# Autodesk Inventor assembly: ASY МОО 001 отстойник осветлитель
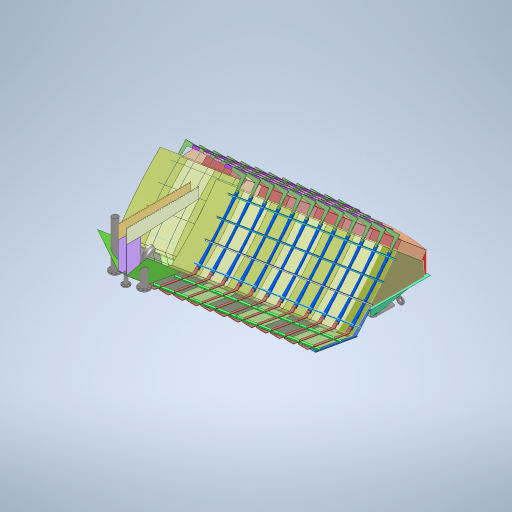
[picture p0: Inventor's stored thumbnail of the model, 512x512]
Saved by Autodesk Inventor 2024.2 (Build 282272000, 272)
## iProperties
Created: 2024-04-28
Part Number: ASY МОО 001 отстойник осветлитель
Document SubType Name: Weldment
Designer: admin
Weld Material: Welded Aluminum-6061
Mass: 1.58517e+06 g
Surface Area: 1.48953e+06 cm^2
Volume: 226523 cm^3
Density: 6.99781 g/cm^3
Author: admin
## Documents named in this file (40)
- C:\Users\pokla\Documents\Inventor\Отстойник осветлитель\Manturovo_Se-clar-Gleb\ASY МОО 001 отстойник осветлитель.iam
- C:\Users\pokla\Documents\Inventor\Отстойник осветлитель\Manturovo_Se-clar-Gleb\МОО 010 лист спина 1.ipt
- C:\Users\pokla\Documents\Inventor\Отстойник осветлитель\Manturovo_Se-clar-Gleb\Пример емкости.ipt
- C:\Users\pokla\Documents\Inventor\Отстойник осветлитель\Manturovo_Se-clar-Gleb\МОО 030 лист брюхо 1.ipt
- C:\Users\pokla\Documents\Inventor\Отстойник осветлитель\Manturovo_Se-clar-Gleb\МОО 040 шпангоут борт 1.ipt
- C:\Users\pokla\Documents\Inventor\Отстойник осветлитель\Manturovo_Se-clar-Gleb\МОО 041 шпангоут спина 1.ipt
- C:\Users\pokla\Documents\Inventor\Отстойник осветлитель\Manturovo_Se-clar-Gleb\Рама основания\ASY МОО 040 рама основания.iam
- C:\Users\pokla\Documents\Inventor\Отстойник осветлитель\Manturovo_Se-clar-Gleb\ASY МОО 060 ракета.iam
- C:\Users\pokla\Documents\Inventor\Отстойник осветлитель\Manturovo_Se-clar-Gleb\Content Center Files\en-US\ISO 5251 B 3D\ISO 5251 Bends 3D without straight ends(90 deg) DN80 2 2.ipt
- C:\Users\pokla\Documents\Inventor\Отстойник осветлитель\Manturovo_Se-clar-Gleb\Content Center Files\en-US\ISO 5251(1)\ISO 5251 Concentric reducers DN80 x DN65 3,2 3,2.ipt
- C:\Users\pokla\Documents\Inventor\Отстойник осветлитель\Manturovo_Se-clar-Gleb\ASY МОО 020 конус.iam
- C:\Users\pokla\Documents\Inventor\Отстойник осветлитель\Manturovo_Se-clar-Gleb\ракета\МОО 064 ракета труба.ipt
- C:\Users\pokla\Documents\Inventor\Отстойник осветлитель\Manturovo_Se-clar-Gleb\х_размеры МОО отстойник осветлитель Dummu.ipt
- C:\Users\pokla\Documents\Inventor\Отстойник осветлитель\Manturovo_Se-clar-Gleb\МОО 012 лист спина 2.ipt
- C:\Users\pokla\Documents\Inventor\Отстойник осветлитель\Manturovo_Se-clar-Gleb\Content Center Files\en-US\DIN EN 1092-1 01 - PN 25\DIN EN 1092-1 Plate Flange for Welding Type 01 - PN 25 80 x 88.9.ipt
- C:\Users\pokla\Documents\Inventor\Отстойник осветлитель\Manturovo_Se-clar-Gleb\МОО 011 лист борт.ipt
- C:\Users\pokla\Documents\Inventor\Отстойник осветлитель\Manturovo_Se-clar-Gleb\Листы бака Глеб\МОО 031 Усилитель спина.ipt
- C:\Users\pokla\Documents\Inventor\Отстойник осветлитель\Manturovo_Se-clar-Gleb\Листы бака Глеб\032 Усилитель левый борт.ipt
- C:\Users\pokla\Documents\Inventor\Отстойник осветлитель\Manturovo_Se-clar-Gleb\МОО 010 лист спина-бедро.ipt
- C:\Users\pokla\Documents\Inventor\Отстойник осветлитель\Manturovo_Se-clar-Gleb\МОО 011 лист борт левый борт бедро.ipt
- C:\Users\pokla\Documents\Inventor\Отстойник осветлитель\Manturovo_Se-clar-Gleb\МОО 011 лист борт правый борт бедро.ipt
- C:\Users\pokla\Documents\Inventor\Отстойник осветлитель\Manturovo_Se-clar-Gleb\МОО 014 лист спина-холка.ipt
- C:\Users\pokla\Documents\Inventor\Отстойник осветлитель\Manturovo_Se-clar-Gleb\МОО 032 лист брюхо-горло.ipt
- C:\Users\pokla\Documents\Inventor\Отстойник осветлитель\Manturovo_Se-clar-Gleb\МОО 035 лист борт.ipt
- C:\Users\pokla\Documents\Inventor\Отстойник осветлитель\Manturovo_Se-clar-Gleb\конус\МОО 051 гребень 1.ipt
- C:\Users\pokla\Documents\Inventor\Отстойник осветлитель\Manturovo_Se-clar-Gleb\конус\МОО 052 гребень 2.ipt
- C:\Users\pokla\Documents\Inventor\Отстойник осветлитель\Manturovo_Se-clar-Gleb\конус\МОО 053 морда 3.ipt
- C:\Users\pokla\Documents\Inventor\Отстойник осветлитель\Manturovo_Se-clar-Gleb\Content Center Files\en-US\ISO 5251 B 3D\ISO 5251 Bends 3D without straight ends(90 deg) DN150 11 11.ipt
- C:\Users\pokla\Documents\Inventor\Отстойник осветлитель\Manturovo_Se-clar-Gleb\Content Center Files\en-US\DIN EN 1092-1 01 - PN 25\DIN EN 1092-1 Plate Flange for Welding Type 01 - PN 25 150 x 168.3.ipt
- C:\Users\pokla\Documents\Inventor\Отстойник осветлитель\Manturovo_Se-clar-Gleb\МОО 061 труба верх 1.ipt
- C:\Users\pokla\Documents\Inventor\Отстойник осветлитель\Manturovo_Se-clar-Gleb\МОО 062 труба верх 2.ipt
- C:\Users\pokla\Documents\Inventor\Отстойник осветлитель\Manturovo_Se-clar-Gleb\МОО 063 труба верх 3.ipt
- C:\Users\pokla\Documents\Inventor\Отстойник осветлитель\Manturovo_Se-clar-Gleb\МОО 051 стрингер спина 1.ipt
- C:\Users\pokla\Documents\Inventor\Отстойник осветлитель\Manturovo_Se-clar-Gleb\МОО 053 стрингер борт 3.ipt
- C:\Users\pokla\Documents\Inventor\Отстойник осветлитель\Manturovo_Se-clar-Gleb\МОО 052 стрингер спина 22.ipt
- C:\Users\pokla\Documents\Inventor\Отстойник осветлитель\Manturovo_Se-clar-Gleb\МОО 054 стрингер борт 43.ipt
- C:\Users\pokla\Documents\Inventor\Отстойник осветлитель\Manturovo_Se-clar-Gleb\МОО 055 стрингер борт 52.ipt
- C:\Users\pokla\Documents\Inventor\Отстойник осветлитель\Manturovo_Se-clar-Gleb\МОО 056 стрингер борт 62.ipt
- C:\Users\pokla\Documents\Inventor\Отстойник осветлитель\Manturovo_Se-clar-Gleb\МОО 057 стрингер борт 7.ipt
- C:\Users\pokla\Documents\Inventor\Отстойник осветлитель\Manturovo_Se-clar-Gleb\МОО 042 шпангоут брюхо.ipt
## Components (191 placed, 40 different names)
1. Пример емкости:1 — Mate:1, Mate:2, Flush:2
2. х_размеры МОО отстойник осветлитель Dummu:1
3. ASY МОО 040 рама основания:1 [sub-assembly] — Flush:19, Flush:20, Flush:21
4. МОО 010 лист спина 1:1 — Flush:3, Rigid:11, Rigid:12
5. МОО 030 лист брюхо 1:1 — Mate:9, Rigid:18, Rigid:40
6. ASY МОО 060 ракета:1 [sub-assembly] — Flush:23, Rigid:10
7. ISO 5251 Bends 3D without straight ends(90 deg) DN80 2:1 — Rigid:2, Rigid:3
8. ISO 5251 Concentric reducers DN80 x DN65 3,2:1 — Rigid:2, Rigid:10
9. ASY МОО 020 конус:1 [sub-assembly] — Flush:22, Mate:16, Flush:28, Mate:31, Mate:36, Mate:54, Mate:57
10. МОО 064 ракета труба:1 — Rigid:3, Cylindrical:1
11. МОО 010 лист спина 1:2 — Rigid:11, Tangent:1, Tangent:3, Rigid:37
12. МОО 010 лист спина 1:3 — Flush:24, Rigid:12, Mate:19, Mate:22, Rigid:30, Mate:31, Flush:44, Tangent:8, Tangent:9
13. МОО 012 лист спина 2:1 — Mate:15, Mate:16, Flush:27, Mate:19, Mate:22
14. DIN EN 1092-1 Plate Flange for Welding Type 01 - PN 25 80 x 88.9:1 — Flush:25, Flush:26, Mate:18, Cylindrical:1
15. МОО 011 лист борт:1 — Flush:30, Tangent:1, Rigid:35, Mate:37
16. МОО 031 Усилитель спина:1
17. 032 Усилитель левый борт:1
18. МОО 030 лист брюхо 1:2 — Rigid:18, Rigid:53
19. МОО 010 лист спина-бедро:1 — Mate:24, Rigid:30, Flush:42, Tangent:6, Flush:43, Tangent:7
20. МОО 011 лист борт левый борт бедро:1 — Flush:41, Flush:42, Tangent:6
21. МОО 011 лист борт правый борт бедро:1 — Mate:30, Flush:43, Tangent:7
22. МОО 011 лист борт:7 — Rigid:35, Rigid:36
23. МОО 011 лист борт:8 — Rigid:36, Rigid:49
24. МОО 010 лист спина 1:5 — Rigid:37, Rigid:38
25. МОО 010 лист спина 1:6 — Rigid:38, Rigid:39
26. МОО 014 лист спина-холка:1 — Rigid:39
27. МОО 030 лист брюхо 1:4 — Rigid:40, Rigid:47
28. МОО 032 лист брюхо-горло:1 — Rigid:48, Mate:52, Mate:53, Rigid:54, Rigid:58, Rigid:61
29. МОО 030 лист брюхо 1:5 — Rigid:45, Rigid:47
30. МОО 030 лист брюхо 1:6 — Rigid:45, Rigid:48
31. МОО 011 лист борт:9 — Rigid:49, Rigid:50
32. МОО 011 лист борт:10 — Rigid:50, Rigid:105
33. МОО 035 лист борт:1 — Mate:36, Flush:47, Tangent:8, Mate:37, Mate:55
34. МОО 051 гребень 1:1 — Mate:50, Mate:56, Flush:48, Rigid:57
35. МОО 052 гребень 2:1 — Rigid:56
36. МОО 053 морда 3:1 — Mate:51, Mate:52, Rigid:52, Mate:53, Mate:56
37. МОО 053 морда 3:2 — Rigid:52, Flush:48
38. МОО 030 лист брюхо 1:7 — Mate:54, Mate:55, Rigid:53
39. DIN EN 1092-1 Plate Flange for Welding Type 01 - PN 25 80 x 88.9:2 — Rigid:54, Rigid:62
40. МОО 051 гребень 1:2 — Rigid:56
41. МОО 052 гребень 2:2 — Rigid:57
42. DIN EN 1092-1 Plate Flange for Welding Type 01 - PN 25 150 x 168.3:1 — Rigid:58, Rotational:1
43. МОО 061 труба верх 1:1 — Rotational:1, Rigid:59
44. ISO 5251 Bends 3D without straight ends(90 deg) DN150 11:1 — Rigid:59
45. МОО 062 труба верх 2:1 — Rigid:60
46. DIN EN 1092-1 Plate Flange for Welding Type 01 - PN 25 150 x 168.3:2 — Rigid:60, Rigid:61
47. МОО 063 труба верх 3:1 — Rigid:62
48. МОО 011 лист борт:11 — Rigid:106
49. МОО 011 лист борт:12
50. МОО 011 лист борт:13
51. МОО 011 лист борт:14
52. МОО 011 лист борт:15 — Rigid:67
53. МОО 035 лист борт:2 — Rigid:67, Mate:57, Mate:58, Tangent:9
54. МОО 011 лист борт:16 — Rigid:105
55. МОО 011 лист борт:17 — Rigid:106
56. МОО 041 шпангоут спина БАЗА 1:2 — Flush:12, Tangent:3, Rigid:25, Flush:44, Rigid:72, Rigid:90, Rigid:92
57. МОО 041 шпангоут спина 1:3 — Rigid:25, Rigid:74, Rigid:91, Rigid:93
58. МОО 040 шпангоут борт 1:1 — Rigid:72, Rigid:88, Rigid:95, Rigid:97, Rigid:99, Rigid:107
59. МОО 042 шпангоут брюхо:1 — Rigid:107, Rigid:109, Rigid:110
60. МОО 042 шпангоут брюхо:2 — Rigid:108, Rigid:111, Rigid:112
61. МОО 040 шпангоут борт 1:2 — Rigid:74, Rigid:94, Rigid:96, Rigid:98, Rigid:100, Rigid:108
62. МОО 041 шпангоут спина 1:4
63. МОО 041 шпангоут спина 1:5
64. МОО 040 шпангоут борт 1:3
65. МОО 042 шпангоут брюхо:3
66. МОО 042 шпангоут брюхо:4
67. МОО 040 шпангоут борт 1:4
68. МОО 041 шпангоут спина 1:6
69. МОО 041 шпангоут спина 1:7
70. МОО 040 шпангоут борт 1:5
71. МОО 042 шпангоут брюхо:5
72. МОО 042 шпангоут брюхо:6
73. МОО 040 шпангоут борт 1:6
74. МОО 041 шпангоут спина 1:8
75. МОО 041 шпангоут спина 1:9
76. МОО 040 шпангоут борт 1:7
77. МОО 042 шпангоут брюхо:7
78. МОО 042 шпангоут брюхо:8
79. МОО 040 шпангоут борт 1:8
80. МОО 041 шпангоут спина 1:10
81. МОО 041 шпангоут спина 1:11
82. МОО 040 шпангоут борт 1:9
83. МОО 042 шпангоут брюхо:9
84. МОО 042 шпангоут брюхо:10
85. МОО 040 шпангоут борт 1:10
86. МОО 041 шпангоут спина 1:12
87. МОО 041 шпангоут спина 1:13
88. МОО 040 шпангоут борт 1:11
89. МОО 042 шпангоут брюхо:11
90. МОО 042 шпангоут брюхо:12
91. МОО 040 шпангоут борт 1:12
92. МОО 041 шпангоут спина 1:14
93. МОО 041 шпангоут спина 1:15
94. МОО 040 шпангоут борт 1:13
95. МОО 042 шпангоут брюхо:13
96. МОО 042 шпангоут брюхо:14
97. МОО 040 шпангоут борт 1:14
98. МОО 041 шпангоут спина 1:16
99. МОО 041 шпангоут спина 1:17
100. МОО 040 шпангоут борт 1:15
101. МОО 042 шпангоут брюхо:15
102. МОО 042 шпангоут брюхо:16
103. МОО 040 шпангоут борт 1:16
104. МОО 041 шпангоут спина 1:18
105. МОО 041 шпангоут спина 1:19
106. МОО 040 шпангоут борт 1:17
107. МОО 042 шпангоут брюхо:17
108. МОО 042 шпангоут брюхо:18
109. МОО 040 шпангоут борт 1:18
110. МОО 041 шпангоут спина 1:20
111. МОО 041 шпангоут спина 1:21
112. МОО 040 шпангоут борт 1:19
113. МОО 042 шпангоут брюхо:19
114. МОО 042 шпангоут брюхо:20
115. МОО 040 шпангоут борт 1:20
116. МОО 041 шпангоут спина 1:22
117. МОО 041 шпангоут спина 1:23
118. МОО 040 шпангоут борт 1:21
119. МОО 042 шпангоут брюхо:21
120. МОО 042 шпангоут брюхо:22
121. МОО 040 шпангоут борт 1:22
122. МОО 041 шпангоут спина 1:24
123. МОО 041 шпангоут спина 1:25
124. МОО 040 шпангоут борт 1:23
125. МОО 042 шпангоут брюхо:23
126. МОО 042 шпангоут брюхо:24
127. МОО 040 шпангоут борт 1:24
128. МОО 052 стрингер спина 2:1 — Rigid:92
129. МОО 051 стрингер спина 1:1 — Rigid:90
130. МОО 051 стрингер спина 1:2 — Rigid:91
131. МОО 052 стрингер спина 2:2 — Rigid:93
132. МОО 053 стрингер борт 3:1 — Rigid:88
133. МОО 054 стрингер борт 4:1 — Rigid:95
134. МОО 055 стрингер борт 5:1 — Rigid:97
135. МОО 056 стрингер борт 6:1 — Rigid:99
136. МОО 057 стрингер борт 7:1 — Rigid:109
137. МОО 057 стрингер борт 7:2 — Rigid:110
138. МОО 053 стрингер борт 3:2 — Rigid:94
139. МОО 054 стрингер борт 4:2 — Rigid:96
140. МОО 055 стрингер борт 5:2 — Rigid:98
141. МОО 056 стрингер борт 6:2 — Rigid:100
142. МОО 057 стрингер борт 7:3 — Rigid:111
143. МОО 057 стрингер борт 7:4 — Rigid:112
144. МОО 052 стрингер спина 2:3
145. МОО 051 стрингер спина 1:3
146. МОО 051 стрингер спина 1:4
147. МОО 052 стрингер спина 2:4
148. МОО 053 стрингер борт 3:3
149. МОО 054 стрингер борт 4:3
150. МОО 055 стрингер борт 5:3
151. МОО 056 стрингер борт 6:3
152. МОО 057 стрингер борт 7:5
153. МОО 057 стрингер борт 7:6
154. МОО 053 стрингер борт 3:4
155. МОО 054 стрингер борт 4:4
156. МОО 055 стрингер борт 5:4
157. МОО 056 стрингер борт 6:4
158. МОО 057 стрингер борт 7:7
159. МОО 057 стрингер борт 7:8
160. МОО 052 стрингер спина 2:5
161. МОО 051 стрингер спина 1:5
162. МОО 051 стрингер спина 1:6
163. МОО 052 стрингер спина 2:6
164. МОО 053 стрингер борт 3:5
165. МОО 054 стрингер борт 4:5
166. МОО 055 стрингер борт 5:5
167. МОО 056 стрингер борт 6:5
168. МОО 057 стрингер борт 7:9
169. МОО 057 стрингер борт 7:10
170. МОО 053 стрингер борт 3:6
171. МОО 054 стрингер борт 4:6
172. МОО 055 стрингер борт 5:6
173. МОО 056 стрингер борт 6:6
174. МОО 057 стрингер борт 7:11
175. МОО 057 стрингер борт 7:12
176. МОО 052 стрингер спина 2:7
177. МОО 051 стрингер спина 1:7
178. МОО 051 стрингер спина 1:8
179. МОО 052 стрингер спина 2:8
180. МОО 053 стрингер борт 3:7
181. МОО 054 стрингер борт 4:7
182. МОО 055 стрингер борт 5:7
183. МОО 056 стрингер борт 6:7
184. МОО 057 стрингер борт 7:13
185. МОО 057 стрингер борт 7:14
186. МОО 053 стрингер борт 3:8
187. МОО 054 стрингер борт 4:8
188. МОО 055 стрингер борт 5:8
189. МОО 056 стрингер борт 6:8
190. МОО 057 стрингер борт 7:15
191. МОО 057 стрингер борт 7:16
## Component patterns: (12 elements, first: МОО 041 шпангоут спина БАЗА 1:2 + МОО 041 шпангоут спина 1:3 + МОО 040 шпангоут борт 1:1 + МОО 042 шпангоут брюхо:1 + МОО 042 шпангоут брюхо:2 + МОО 040 шпангоут борт 1:2), (4 elements, first: МОО 052 стрингер спина 2:1 + МОО 051 стрингер спина 1:1 + МОО 051 стрингер спина 1:2 + МОО 052 стрингер спина 2:2 + МОО 053 стрингер борт 3:1 + МОО 054 стрингер борт 4:1 + МОО 055 стрингер борт 5:1 + МОО 056 стрингер борт 6:1 + МОО 057 стрингер борт 7:1 + МОО 057 стрингер борт 7:2 + МОО 053 стрингер борт 3:2 + МОО 054 стрингер борт 4:2 + МОО 055 стрингер борт 5:2 + МОО 056 стрингер борт 6:2 + МОО 057 стрингер борт 7:3 + МОО 057 стрингер борт 7:4)
## Relationships (106: WeldJoint 56, Mate 22, Flush 20, Tangent 6, CylindricalJoint 1, RevoluteJoint 1)
- Mate:1: Пример емкости:1
- Mate:2: Пример емкости:1
- Flush:2: Пример емкости:1
- Flush:3: МОО 010 лист спина 1:1
- Mate:9: МОО 030 лист брюхо 1:1
- Flush:12: МОО 041 шпангоут спина БАЗА 1:2
- Rigid:2 [WeldJoint]: ISO 5251 Bends 3D without straight ends(90 deg) DN80 2:1 ↔ ISO 5251 Concentric reducers DN80 x DN65 3,2:1
- Rigid:3 [WeldJoint]: ISO 5251 Bends 3D without straight ends(90 deg) DN80 2:1 ↔ МОО 064 ракета труба:1
- Flush:19 (-250 mm): ASY МОО 040 рама основания:1
- Flush:20: ASY МОО 040 рама основания:1
- Flush:21: ASY МОО 040 рама основания:1
- Flush:22: ASY МОО 020 конус:1
- Flush:23: ASY МОО 060 ракета:1
- Mate:15: МОО 012 лист спина 2:1
- Flush:24: МОО 010 лист спина 1:3
- Mate:16: ASY МОО 020 конус:1 ↔ МОО 012 лист спина 2:1
- Flush:25: DIN EN 1092-1 Plate Flange for Welding Type 01 - PN 25 80 x 88.9:1
- Flush:26: DIN EN 1092-1 Plate Flange for Welding Type 01 - PN 25 80 x 88.9:1
- Mate:18 (120 mm): DIN EN 1092-1 Plate Flange for Welding Type 01 - PN 25 80 x 88.9:1
- Rigid:10 [WeldJoint] (-20 mm): ASY МОО 060 ракета:1 ↔ ISO 5251 Concentric reducers DN80 x DN65 3,2:1
- Cylindrical:1: МОО 064 ракета труба:1 ↔ DIN EN 1092-1 Plate Flange for Welding Type 01 - PN 25 80 x 88.9:1
- Flush:27 (15 mm): МОО 012 лист спина 2:1
- Flush:28: ASY МОО 020 конус:1
- Rigid:11 [WeldJoint]: МОО 010 лист спина 1:1 ↔ МОО 010 лист спина 1:2
- Rigid:12 [WeldJoint]: МОО 010 лист спина 1:1 ↔ МОО 010 лист спина 1:3
- Mate:19 (910 mm): МОО 010 лист спина 1:3 ↔ МОО 012 лист спина 2:1
- Flush:30: МОО 011 лист борт:1
- Tangent:1: МОО 010 лист спина 1:2 ↔ МОО 011 лист борт:1
- Tangent:3: МОО 010 лист спина 1:2 ↔ МОО 041 шпангоут спина БАЗА 1:2
- Mate:22 (47 mm): МОО 010 лист спина 1:3 ↔ МОО 012 лист спина 2:1
- Rigid:18 [WeldJoint]: МОО 030 лист брюхо 1:1 ↔ МОО 030 лист брюхо 1:2
- Rigid:25 [WeldJoint] (-50 mm): МОО 041 шпангоут спина БАЗА 1:2 ↔ МОО 041 шпангоут спина 1:3
- Mate:24: МОО 010 лист спина-бедро:1
- Rigid:30 [WeldJoint]: МОО 010 лист спина 1:3 ↔ МОО 010 лист спина-бедро:1
- Flush:41: МОО 011 лист борт левый борт бедро:1
- Flush:42: МОО 010 лист спина-бедро:1 ↔ МОО 011 лист борт левый борт бедро:1
- Tangent:6: МОО 010 лист спина-бедро:1 ↔ МОО 011 лист борт левый борт бедро:1
- Mate:30: МОО 011 лист борт правый борт бедро:1
- Flush:43: МОО 010 лист спина-бедро:1 ↔ МОО 011 лист борт правый борт бедро:1
- Tangent:7: МОО 010 лист спина-бедро:1 ↔ МОО 011 лист борт правый борт бедро:1
- Rigid:35 [WeldJoint]: МОО 011 лист борт:1 ↔ МОО 011 лист борт:7
- Rigid:36 [WeldJoint]: МОО 011 лист борт:7 ↔ МОО 011 лист борт:8
- Rigid:37 [WeldJoint]: МОО 010 лист спина 1:2 ↔ МОО 010 лист спина 1:5
- Rigid:38 [WeldJoint]: МОО 010 лист спина 1:5 ↔ МОО 010 лист спина 1:6
- Rigid:39 [WeldJoint]: МОО 010 лист спина 1:6 ↔ МОО 014 лист спина-холка:1
- Mate:31: ASY МОО 020 конус:1 ↔ МОО 010 лист спина 1:3
- Rigid:40 [WeldJoint]: МОО 030 лист брюхо 1:1 ↔ МОО 030 лист брюхо 1:4
- Flush:44 (-250 mm): МОО 010 лист спина 1:3 ↔ МОО 041 шпангоут спина БАЗА 1:2
- Rigid:45 [WeldJoint]: МОО 030 лист брюхо 1:5 ↔ МОО 030 лист брюхо 1:6
- Rigid:47 [WeldJoint]: МОО 030 лист брюхо 1:4 ↔ МОО 030 лист брюхо 1:5
- Rigid:48 [WeldJoint]: МОО 032 лист брюхо-горло:1 ↔ МОО 030 лист брюхо 1:6
- Rigid:49 [WeldJoint]: МОО 011 лист борт:8 ↔ МОО 011 лист борт:9
- Rigid:50 [WeldJoint]: МОО 011 лист борт:9 ↔ МОО 011 лист борт:10
- Mate:36: ASY МОО 020 конус:1 ↔ МОО 035 лист борт:1
- Flush:47: МОО 035 лист борт:1
- Tangent:8: МОО 010 лист спина 1:3 ↔ МОО 035 лист борт:1
- Mate:37: МОО 011 лист борт:1 ↔ МОО 035 лист борт:1
- Mate:50 (110 mm): МОО 051 гребень 1:1
- Mate:51: МОО 053 морда 3:1
- Mate:52: МОО 032 лист брюхо-горло:1 ↔ МОО 053 морда 3:1
- Rigid:52 [WeldJoint]: МОО 053 морда 3:1 ↔ МОО 053 морда 3:2
- Mate:53 (-10 mm): МОО 032 лист брюхо-горло:1 ↔ МОО 053 морда 3:1
- Mate:54: ASY МОО 020 конус:1 ↔ МОО 030 лист брюхо 1:7
- Mate:55: МОО 035 лист борт:1 ↔ МОО 030 лист брюхо 1:7
- Rigid:53 [WeldJoint]: МОО 030 лист брюхо 1:2 ↔ МОО 030 лист брюхо 1:7
- Mate:56: МОО 051 гребень 1:1 ↔ МОО 053 морда 3:1
- Rigid:54 [WeldJoint] (200 mm): МОО 032 лист брюхо-горло:1 ↔ DIN EN 1092-1 Plate Flange for Welding Type 01 - PN 25 80 x 88.9:2
- Flush:48 (-50 mm): МОО 051 гребень 1:1 ↔ МОО 053 морда 3:2
- Rigid:56 [WeldJoint]: МОО 052 гребень 2:1 ↔ МОО 051 гребень 1:2
- Rigid:57 [WeldJoint]: МОО 051 гребень 1:1 ↔ МОО 052 гребень 2:2
- Rigid:58 [WeldJoint] (300 mm): МОО 032 лист брюхо-горло:1 ↔ DIN EN 1092-1 Plate Flange for Welding Type 01 - PN 25 150 x 168.3:1
- Rotational:1 [RevoluteJoint]: DIN EN 1092-1 Plate Flange for Welding Type 01 - PN 25 150 x 168.3:1 ↔ МОО 061 труба верх 1:1
- Rigid:59 [WeldJoint]: МОО 061 труба верх 1:1 ↔ ISO 5251 Bends 3D without straight ends(90 deg) DN150 11:1
- Rigid:60 [WeldJoint]: МОО 062 труба верх 2:1 ↔ DIN EN 1092-1 Plate Flange for Welding Type 01 - PN 25 150 x 168.3:2
- Rigid:61 [WeldJoint] (300 mm): МОО 032 лист брюхо-горло:1 ↔ DIN EN 1092-1 Plate Flange for Welding Type 01 - PN 25 150 x 168.3:2
- Rigid:62 [WeldJoint]: DIN EN 1092-1 Plate Flange for Welding Type 01 - PN 25 80 x 88.9:2 ↔ МОО 063 труба верх 3:1
- [WeldJoint]: МОО 011 лист борт:11 ↔ МОО 011 лист борт:12
- [WeldJoint]: МОО 011 лист борт:12 ↔ МОО 011 лист борт:13
- [WeldJoint]: МОО 011 лист борт:13 ↔ МОО 011 лист борт:14
- [WeldJoint]: МОО 011 лист борт:14 ↔ МОО 011 лист борт:15
- Rigid:67 [WeldJoint]: МОО 011 лист борт:15 ↔ МОО 035 лист борт:2
- Mate:57: ASY МОО 020 конус:1 ↔ МОО 035 лист борт:2
- Mate:58: МОО 035 лист борт:2
- Tangent:9: МОО 010 лист спина 1:3 ↔ МОО 035 лист борт:2
- Rigid:72 [WeldJoint] (-50 mm): МОО 041 шпангоут спина БАЗА 1:2 ↔ МОО 040 шпангоут борт 1:1
- Rigid:74 [WeldJoint] (-50 mm): МОО 041 шпангоут спина 1:3 ↔ МОО 040 шпангоут борт 1:2
- Rigid:88 [WeldJoint] (2 mm): МОО 040 шпангоут борт 1:1 ↔ МОО 053 стрингер борт 3:1
- Rigid:90 [WeldJoint] (2 mm): МОО 041 шпангоут спина БАЗА 1:2 ↔ МОО 051 стрингер спина 1:1
- Rigid:91 [WeldJoint] (2 mm): МОО 041 шпангоут спина 1:3 ↔ МОО 051 стрингер спина 1:2
- Rigid:92 [WeldJoint] (2 mm): МОО 041 шпангоут спина БАЗА 1:2 ↔ МОО 052 стрингер спина 2:1
- Rigid:93 [WeldJoint] (2 mm): МОО 041 шпангоут спина 1:3 ↔ МОО 052 стрингер спина 2:2
- Rigid:94 [WeldJoint] (2 mm): МОО 040 шпангоут борт 1:2 ↔ МОО 053 стрингер борт 3:2
- Rigid:95 [WeldJoint] (2 mm): МОО 040 шпангоут борт 1:1 ↔ МОО 054 стрингер борт 4:1
- Rigid:96 [WeldJoint] (2 mm): МОО 040 шпангоут борт 1:2 ↔ МОО 054 стрингер борт 4:2
- Rigid:97 [WeldJoint] (2 mm): МОО 040 шпангоут борт 1:1 ↔ МОО 055 стрингер борт 5:1
- Rigid:98 [WeldJoint] (2 mm): МОО 040 шпангоут борт 1:2 ↔ МОО 055 стрингер борт 5:2
- Rigid:99 [WeldJoint] (2 mm): МОО 040 шпангоут борт 1:1 ↔ МОО 056 стрингер борт 6:1
- Rigid:100 [WeldJoint] (2 mm): МОО 040 шпангоут борт 1:2 ↔ МОО 056 стрингер борт 6:2
- Rigid:105 [WeldJoint]: МОО 011 лист борт:10 ↔ МОО 011 лист борт:16
- Rigid:106 [WeldJoint]: МОО 011 лист борт:11 ↔ МОО 011 лист борт:17
- Rigid:107 [WeldJoint] (-50 mm): МОО 040 шпангоут борт 1:1 ↔ МОО 042 шпангоут брюхо:1
- Rigid:108 [WeldJoint] (-50 mm): МОО 042 шпангоут брюхо:2 ↔ МОО 040 шпангоут борт 1:2
- Rigid:109 [WeldJoint] (2 mm): МОО 042 шпангоут брюхо:1 ↔ МОО 057 стрингер борт 7:1
- Rigid:110 [WeldJoint] (2 mm): МОО 042 шпангоут брюхо:1 ↔ МОО 057 стрингер борт 7:2
- Rigid:111 [WeldJoint] (2 mm): МОО 042 шпангоут брюхо:2 ↔ МОО 057 стрингер борт 7:3
- Rigid:112 [WeldJoint] (2 mm): МОО 042 шпангоут брюхо:2 ↔ МОО 057 стрингер борт 7:4
## Named parameters: Бак_нахлест_фланца = 25 mm, d230_d194 = 0 mm, d231_d195 = 0 mm, d232_d160 = 0 mm, d233_d161 = 0 mm
